# Autodesk Inventor assembly: bumper
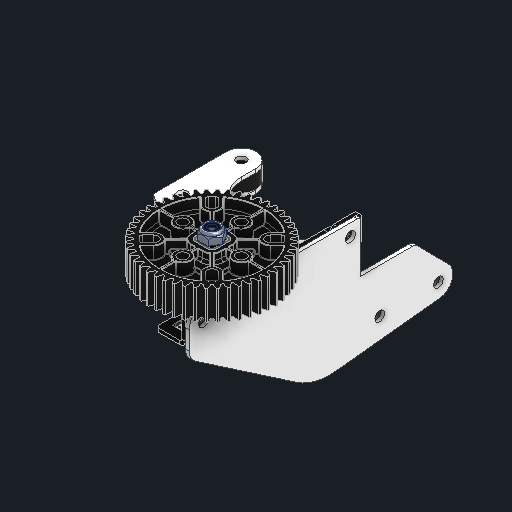
[picture p0: Inventor's stored thumbnail of the model, 512x512]
Saved by Autodesk Inventor 2024 (Build 280153000, 153)
## iProperties
Created: 2024-02-11
Part Number: bumper
Document SubType Name: Assembly
Designer: Averey Ku
Author: Averey Ku
## Documents named in this file (16)
- D:\vex_robotics\hardware\cad\vroomba_v0.1\chassis\drivebay\bumper.iam
- D:\vex_robotics\hardware\cad\vroomba_v0.1\custom_parts\drivebay\gusset.ipt
- D:\vex_robotics\hardware\cad\VEX-CAD-Inventor-1.41\Motion\Spacers\Spacer Nylon .500 OD\NSpacer Black .500 OD x .250.ipt
- D:\vex_robotics\hardware\cad\VEX-CAD-Inventor-1.41\Motion\Spacers\Spacer Nylon .500 OD.ipt
- D:\vex_robotics\hardware\cad\VEX-CAD-Inventor-1.41\Structure\Angle\Aluminum 1x1\Alu Angle 1x1x6.ipt
- D:\vex_robotics\hardware\cad\VEX-CAD-Inventor-1.41\Structure\Hardware\Nut Keps.ipt
- D:\vex_robotics\hardware\cad\VEX-CAD-Inventor-1.41\Motion\Spacers\Spacer Nylon .375 OD.ipt
- D:\vex_robotics\hardware\cad\VEX-CAD-Inventor-1.41\Motion\Spacers\Spacer Nylon .375 OD\NSpacer .375 OD x .375.ipt
- D:\vex_robotics\hardware\cad\VEX-CAD-Inventor-1.41\Motion\Gears\HS Gear\HS 48T Gear, No Insert.iam
- D:\vex_robotics\hardware\cad\VEX-CAD-Inventor-1.41\Motion\Gears\HS Gear.iam
- D:\vex_robotics\hardware\cad\VEX-CAD-Inventor-1.41\Structure\Hardware\Nut Thin Nylock.ipt
- D:\vex_robotics\hardware\cad\vroomba_v0.1\custom_parts\drivebay\sled.ipt
- D:\vex_robotics\hardware\cad\VEX-CAD-Inventor-1.41\Motion\Spacers\Washer Teflon\TWasher .375 OD x .04000.ipt
- D:\vex_robotics\hardware\cad\VEX-CAD-Inventor-1.41\Motion\Spacers\Washer Teflon.ipt
- D:\vex_robotics\hardware\cad\VEX-CAD-Inventor-1.41\Motion\Spacers\Washer Steel\SWasher .375 OD x .062500.ipt
- D:\vex_robotics\hardware\cad\VEX-CAD-Inventor-1.41\Motion\Spacers\Washer Steel.ipt
## Components (21 placed, 10 different names)
1. gusset:1 — Insert:1, Insert:2, Insert:3, Insert:4, Insert:6, Insert:7, Insert:8
2. gusset:2 — Insert:5, Mate:1, Insert:9, Mate:2
3. NSpacer Black .500 OD x .250:1 — Insert:1
4. NSpacer Black .500 OD x .250:2 — Insert:2
5. NSpacer Black .500 OD x .250:3 — Insert:3, Mate:1
6. NSpacer Black .500 OD x .250:4 — Insert:4, Insert:5
7. NSpacer Black .500 OD x .250:5 — Insert:7
8. NSpacer Black .500 OD x .250:6 — Insert:6
9. NSpacer Black .500 OD x .250:7 — Insert:8
10. Alu Angle 1x1x6:1 — Insert:9, Mate:2, Insert:10, Insert:14, Mate:3
11. Nut Keps:1 — Insert:10, Insert:11
12. NSpacer .375 OD x .375:1 — Insert:11, Insert:12
13. HS 48T Gear, No Insert:1 [sub-assembly] — Insert:12, Insert:13
14. Nut Thin Nylock:1 — Insert:13
15. sled:1 — Insert:14, Mate:3, Insert:17, Insert:20
16. SWasher .375 OD x .062500:1 — Insert:16, Insert:17
17. TWasher .375 OD x .04000:1 — Insert:15
18. TWasher .375 OD x .04000:2 — Insert:15, Insert:16
19. SWasher .375 OD x .062500:2 — Insert:20
20. TWasher .375 OD x .04000:3
21. TWasher .375 OD x .04000:4
## Relationships (23: Insert 20, Mate 3)
- Insert:1: gusset:1 ↔ NSpacer Black .500 OD x .250:1
- Insert:2: gusset:1 ↔ NSpacer Black .500 OD x .250:2
- Insert:3: gusset:1 ↔ NSpacer Black .500 OD x .250:3
- Insert:4: gusset:1 ↔ NSpacer Black .500 OD x .250:4
- Insert:5: gusset:2 ↔ NSpacer Black .500 OD x .250:4
- Mate:1: gusset:2 ↔ NSpacer Black .500 OD x .250:3
- Insert:6: gusset:1 ↔ NSpacer Black .500 OD x .250:6
- Insert:7: gusset:1 ↔ NSpacer Black .500 OD x .250:5
- Insert:8: gusset:1 ↔ NSpacer Black .500 OD x .250:7
- Insert:9: gusset:2 ↔ Alu Angle 1x1x6:1
- Mate:2: gusset:2 ↔ Alu Angle 1x1x6:1
- Insert:10: Alu Angle 1x1x6:1 ↔ Nut Keps:1
- Insert:11: Nut Keps:1 ↔ NSpacer .375 OD x .375:1
- Insert:12: NSpacer .375 OD x .375:1 ↔ HS 48T Gear, No Insert:1
- Insert:13: HS 48T Gear, No Insert:1 ↔ Nut Thin Nylock:1
- Insert:14: Alu Angle 1x1x6:1 ↔ sled:1
- Mate:3: Alu Angle 1x1x6:1 ↔ sled:1
- Insert:15: TWasher .375 OD x .04000:1 ↔ TWasher .375 OD x .04000:2
- Insert:16: SWasher .375 OD x .062500:1 ↔ TWasher .375 OD x .04000:2
- Insert:17: sled:1 ↔ SWasher .375 OD x .062500:1
- [Insert]: TWasher .375 OD x .04000:3 ↔ TWasher .375 OD x .04000:4
- [Insert]: SWasher .375 OD x .062500:2 ↔ TWasher .375 OD x .04000:4
- Insert:20: sled:1 ↔ SWasher .375 OD x .062500:2
## Named parameters: d25_d22 = 0 mm, d26_d23 = 0 mm
